# Autodesk Inventor assembly: Gantry Table With Chucks - V2
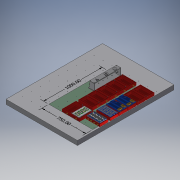
[picture p0: Inventor's stored thumbnail of the model, 180x180]
Saved by Autodesk Inventor 2019.4 (Build 234330000, 330)
## iProperties
Created: 2021-03-04
Part Number: Gantry Table With Chucks - V2
Document SubType Name: Assembly
Designer: caleb
Author: caleb
## Documents named in this file (12)
- C:\Users\cfang\Desktop\nebraska-silicon-lab\Hardware\ETL\Module Assembly\Gantry Table With Chucks - V2.iam
- C:\Users\cfang\Desktop\nebraska-silicon-lab\Hardware\ETL\Module Assembly\Gantry Base.ipt
- C:\Users\cfang\Desktop\nebraska-silicon-lab\Hardware\ETL\Module Assembly\Chuck - V2\Chuck - V2.ipt
- C:\Users\cfang\Desktop\nebraska-silicon-lab\Hardware\General Gantry\Gantry Tool Rack\Tool Rack Assembly.iam
- C:\Users\cfang\Desktop\nebraska-silicon-lab\Hardware\ETL\Module Assembly\Chuck - V2\Chuck - V2.iam
- C:\Users\cfang\Desktop\nebraska-silicon-lab\Hardware\ETL\Module Assembly\Chuck - Octopocket\Chuck - Octopocket.iam
- C:\Users\cfang\Desktop\nebraska-silicon-lab\Hardware\ETL\Module Assembly\BBM Staging Plate\BBM Staging Plate Assembly.iam
- C:\Users\cfang\Desktop\nebraska-silicon-lab\Hardware\ETL\Module Assembly\Glue Reservoir Plate\Glue Reservoir Plate.ipt
- C:\Users\cfang\Desktop\nebraska-silicon-lab\Hardware\ETL\Module Assembly\Glue Stamp Staging Plate\Glue Stamp Staging Plate Assembly.iam
- C:\Users\cfang\Desktop\nebraska-silicon-lab\Hardware\ETL\Module Assembly\Assembly Plate\Assembly Plate Assembly.iam
- C:\Users\cfang\Desktop\nebraska-silicon-lab\Hardware\ETL\Module Assembly\Grabber Tool\Grabber Tool.iam
- C:\Users\cfang\Desktop\nebraska-silicon-lab\Hardware\ETL\Module Assembly\Picker Tool\Picker Tool.iam
## Components (23 placed, 10 different names)
1. Gantry Base:1 — Mate:14, Angle:9, Mate:15, Angle:10, Insert:1, Mate:16, Angle:11, Insert:2, Mate:17, Mate:18, Mate:19, Angle:12, Angle:13, Insert:4, Insert:7, Insert:8
2. Chuck - V2:7
3. Tool Rack Assembly:1 [sub-assembly] — Mate:14, Angle:9, Angle:20, Angle:21, Angle:22, Angle:23, Insert:9, Insert:10
4. Chuck - Octopocket:1 [sub-assembly] — Mate:17, Insert:7, Mate:22, Angle:16
5. Chuck - V2:24 [sub-assembly] — Mate:18, Angle:12, Insert:8, Mate:26
6. Chuck - V2:25 [sub-assembly] — Mate:19, Angle:13, Insert:4
7. BBM Staging Plate Assembly:1 [sub-assembly] — Mate:22, Angle:16
8. Glue Reservoir Plate:1 — Mate:23, Angle:17
9. Glue Stamp Staging Plate Assembly:1 [sub-assembly] — Mate:24, Angle:18
10. Glue Stamp Staging Plate Assembly:2 [sub-assembly] — Mate:25, Angle:19
11. Assembly Plate Assembly:1 [sub-assembly] — Mate:26
12. Grabber Tool:1 [sub-assembly] — Angle:21, Angle:23, Insert:9
13. Picker Tool:1 [sub-assembly] — Angle:20, Angle:22, Insert:10
14. Chuck - V2:13 [sub-assembly] — Mate:15, Angle:10, Insert:1
15. Chuck - V2:14 [sub-assembly]
16. Chuck - V2:15 [sub-assembly]
17. Chuck - V2:16 [sub-assembly]
18. Chuck - V2:17 [sub-assembly]
19. Chuck - V2:19 [sub-assembly] — Mate:16, Angle:11, Insert:2
20. Chuck - V2:20 [sub-assembly]
21. Chuck - V2:21 [sub-assembly] — Mate:25, Angle:19
22. Chuck - V2:22 [sub-assembly] — Mate:24, Angle:18
23. Chuck - V2:23 [sub-assembly] — Mate:23, Angle:17
## Component patterns: (5 elements, first: Chuck - V2:13), (5 elements, first: Chuck - V2:19)
## Relationships (31: Angle 13, Mate 11, Insert 7)
- Mate:14: Gantry Base:1 ↔ Tool Rack Assembly:1
- Angle:9 (0 deg): Gantry Base:1 ↔ Tool Rack Assembly:1
- Mate:15: Gantry Base:1 ↔ Chuck - V2:13
- Angle:10 (0 deg): Gantry Base:1 ↔ Chuck - V2:13
- Insert:1: Gantry Base:1 ↔ Chuck - V2:13
- Mate:16: Gantry Base:1 ↔ Chuck - V2:19
- Angle:11 (0 deg): Gantry Base:1 ↔ Chuck - V2:19
- Insert:2: Gantry Base:1 ↔ Chuck - V2:19
- Mate:17: Gantry Base:1 ↔ Chuck - Octopocket:1
- Mate:18: Gantry Base:1 ↔ Chuck - V2:24
- Mate:19: Gantry Base:1 ↔ Chuck - V2:25
- Angle:12 (0 deg): Gantry Base:1 ↔ Chuck - V2:24
- Angle:13 (0 deg): Gantry Base:1 ↔ Chuck - V2:25
- Insert:4: Gantry Base:1 ↔ Chuck - V2:25
- Insert:7: Gantry Base:1 ↔ Chuck - Octopocket:1
- Insert:8: Gantry Base:1 ↔ Chuck - V2:24
- Mate:22: Chuck - Octopocket:1 ↔ BBM Staging Plate Assembly:1
- Angle:16 (0 deg): Chuck - Octopocket:1 ↔ BBM Staging Plate Assembly:1
- Mate:23: Glue Reservoir Plate:1 ↔ Chuck - V2:23
- Mate:24: Glue Stamp Staging Plate Assembly:1 ↔ Chuck - V2:22
- Mate:25: Glue Stamp Staging Plate Assembly:2 ↔ Chuck - V2:21
- Mate:26: Chuck - V2:24 ↔ Assembly Plate Assembly:1
- Angle:17 (0 deg): Glue Reservoir Plate:1 ↔ Chuck - V2:23
- Angle:18 (0 deg): Glue Stamp Staging Plate Assembly:1 ↔ Chuck - V2:22
- Angle:19 (0 deg): Glue Stamp Staging Plate Assembly:2 ↔ Chuck - V2:21
- Angle:20 (90 deg): Tool Rack Assembly:1 ↔ Picker Tool:1
- Angle:21 (0 deg): Tool Rack Assembly:1 ↔ Grabber Tool:1
- Angle:22 (0 deg): Tool Rack Assembly:1 ↔ Picker Tool:1
- Angle:23 (0 deg): Tool Rack Assembly:1 ↔ Grabber Tool:1
- Insert:9: Tool Rack Assembly:1 ↔ Grabber Tool:1
- Insert:10: Tool Rack Assembly:1 ↔ Picker Tool:1
